# Autodesk Inventor assembly: _Tooling_PCBPaste
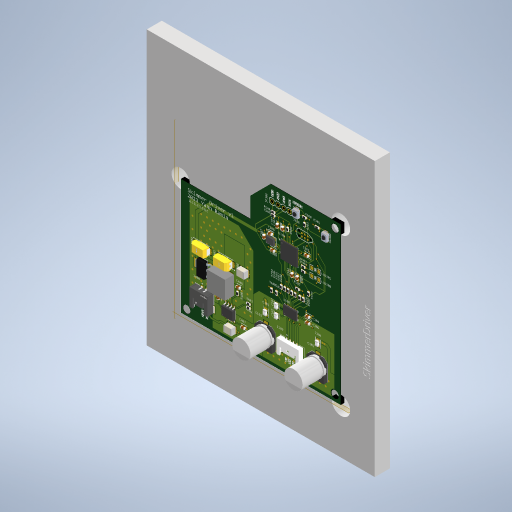
[picture p0: Inventor's stored thumbnail of the model, 512x512]
Saved by Autodesk Inventor 2023.2 (Build 272271000, 271)
## iProperties
Created: 2023-03-08
Part Number: _Tooling_PCBPaste
Document SubType Name: Assembly
Designer: atrus
Author: atrus
## Documents named in this file (3)
- C:\Users\atrus\Dropbox\elec\Mechanical\SkimmerSwabbie\_Tooling_PCBPaste.iam
- C:\Users\atrus\Dropbox\elec\Mechanical\SkimmerSwabbie\PCB\skimmer_swabbie_v1\skimmer_swabbie_v1.iam
- C:\Users\atrus\Dropbox\elec\Mechanical\SkimmerSwabbie\_Tooling_PCBPaste.ipt
## Components (2 placed, 2 different names)
1. skimmer_swabbie_v1:1 [sub-assembly] — Mate:1, Mate:2, Mate:3
2. _Tooling_PCBPaste:1 — Mate:1, Mate:2, Mate:3
## Relationships (3: Mate 3)
- Mate:1: skimmer_swabbie_v1:1 ↔ _Tooling_PCBPaste:1
- Mate:2 (15 mm): skimmer_swabbie_v1:1 ↔ _Tooling_PCBPaste:1
- Mate:3 (20 mm): skimmer_swabbie_v1:1 ↔ _Tooling_PCBPaste:1
